# Autodesk Inventor assembly: Spacer
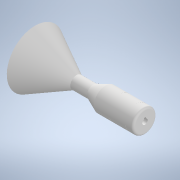
[picture p0: Inventor's stored thumbnail of the model, 180x180]
Saved by Autodesk Inventor 2021.2 (Build 252289000, 289)
## iProperties
Created: 2021-05-18
Part Number: Spacer
Document SubType Name: Assembly
Designer: Ryan
Author: Ryan
## Documents named in this file (4)
- C:\Users\Ryan\Documents\EDD\__NewCompressor\Spacer\Spacer.iam
- C:\Users\Ryan\Documents\EDD\__NewCompressor\Spacer\SpacerA.ipt
- C:\Users\Ryan\Documents\EDD\__NewCompressor\Spacer\SpacerB.ipt
- C:\Users\Ryan\Documents\EDD\__NewCompressor\Spacer\SpacerC.ipt
## Components (3 placed, 3 different names)
1. SpacerA:1 — Insert:1
2. SpacerB:1 — Insert:1, Insert:2
3. SpacerC:1 — Insert:2
## Relationships (2: Insert 2)
- Insert:1: SpacerA:1 ↔ SpacerB:1
- Insert:2: SpacerB:1 ↔ SpacerC:1
